# Autodesk Inventor assembly: final_carrera
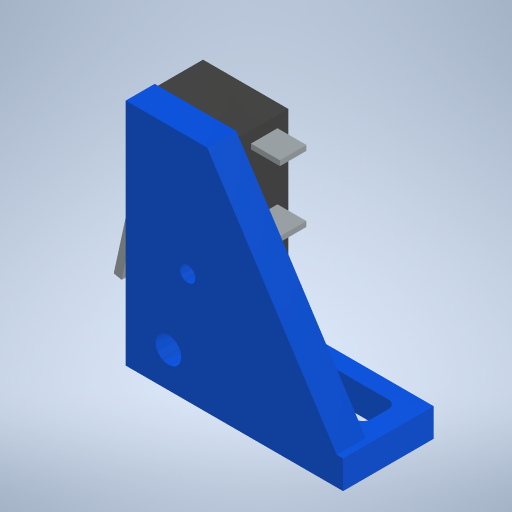
[picture p0: Inventor's stored thumbnail of the model, 512x512]
Saved by Autodesk Inventor 2024.3 (Build 283343000, 343)
## iProperties
Created: 2024-09-30
Part Number: final_carrera
Document SubType Name: Assembly
Designer: User
Author: User
## Documents named in this file (3)
- C:\Users\User\Documents\Universidad Octavo Semestre\Robotica Industrial\matlab\SCARA\mariana_scara_final\mariana_scara_final\final_carrera.iam
- C:\Users\User\Documents\Universidad Octavo Semestre\Robotica Industrial\matlab\SCARA\mariana_scara_final\mariana_scara_final\soporte_final_1.ipt
- C:\Users\User\Documents\Universidad Octavo Semestre\Robotica Industrial\matlab\SCARA\mariana_scara_final\mariana_scara_final\final_2.ipt
## Components (2 placed, 2 different names)
1. soporte_final_1:1 — Mate:1, Flush:1, Mate:2
2. final_2:1 — Mate:1, Flush:1, Mate:2
## Relationships (3: Mate 2, Flush 1)
- Mate:1: soporte_final_1:1 ↔ final_2:1
- Flush:1: soporte_final_1:1 ↔ final_2:1
- Mate:2: soporte_final_1:1 ↔ final_2:1
